# Autodesk Inventor assembly: Assy_cam_connection
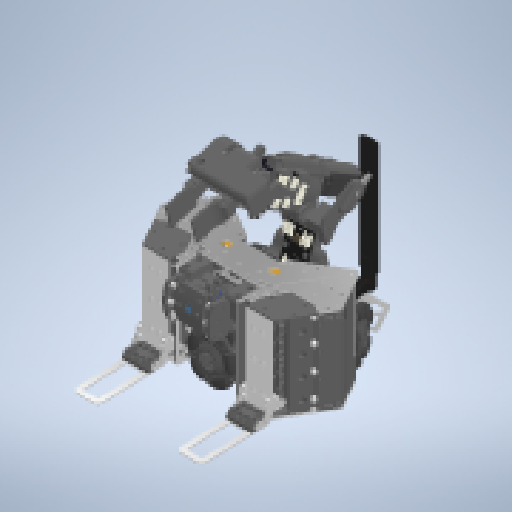
[picture p0: Inventor's stored thumbnail of the model, 512x512]
Saved by Autodesk Inventor 2024.1 (Build 281209000, 209)
## iProperties
Created: 2025-05-03
Part Number: Assy_cam_connection
Document SubType Name: Assembly
Designer: hibik
Author: hibik
## Documents named in this file (7)
- C:\Users\hibik\Documents\Robomech\RESCUE\ORCA\hard\Assy_cam_connection.iam
- C:\Users\hibik\Documents\Robomech\RESCUE\ORCA\hard\Assy_arm_connection.iam
- C:\Users\hibik\Documents\Robomech\RESCUE\ORCA\hard\camera\Assy_camera.iam
- C:\Users\hibik\Documents\Robomech\RESCUE\ORCA\hard\flame_front\cam_setter_right_under.ipt
- C:\Users\hibik\Documents\Robomech\RESCUE\ORCA\hard\flame_front\cam_setter_right_upper.ipt
- C:\Users\hibik\Documents\Robomech\RESCUE\ORCA\hard\flame_front\cam_setter_right_under_MIR.ipt
- C:\Users\hibik\Documents\Robomech\RESCUE\ORCA\hard\flame_front\cam_setter_right_upper_MIR.ipt
## Components (6 placed, 6 different names)
1. Assy_arm_connection:1 [sub-assembly] — 挿入:6, 角度:2
2. Assy_camera:1 [sub-assembly] — 挿入:5, 角度:1
3. cam_setter_right_under:1 — 挿入:1, 挿入:2, 挿入:6
4. cam_setter_right_upper:1 — 挿入:1, 挿入:2, 挿入:5, 角度:1, 角度:2
5. cam_setter_right_under_MIR:1 — 挿入:7, 挿入:8
6. cam_setter_right_upper_MIR:1 — 挿入:7, 挿入:8
## Relationships (8: Insert 6, Angle 2)
- 挿入:1 [Insert]: cam_setter_right_under:1 ↔ cam_setter_right_upper:1
- 挿入:2 [Insert]: cam_setter_right_under:1 ↔ cam_setter_right_upper:1
- 挿入:5 [Insert]: Assy_camera:1 ↔ cam_setter_right_upper:1
- 角度:1 [Angle] (0 deg): Assy_camera:1 ↔ cam_setter_right_upper:1
- 挿入:6 [Insert]: Assy_arm_connection:1 ↔ cam_setter_right_under:1
- 角度:2 [Angle] (0 deg): Assy_arm_connection:1 ↔ cam_setter_right_upper:1
- 挿入:7 [Insert]: cam_setter_right_under_MIR:1 ↔ cam_setter_right_upper_MIR:1
- 挿入:8 [Insert]: cam_setter_right_under_MIR:1 ↔ cam_setter_right_upper_MIR:1
